# Autodesk Inventor assembly: DPLX_A005_Spark_Gap_Lab
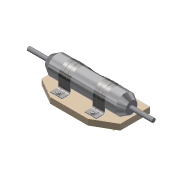
[picture p0: Inventor's stored thumbnail of the model, 180x180]
Saved by Autodesk Inventor 2018 (Build 220112000, 112)
## iProperties
Created: 2018-07-20
Part Number: DPLX_A005_Spark_Gap_Lab
Document SubType Name: Assembly
Designer: DPLXuser
Author: DPLXuser
## Documents named in this file (14)
- C:\Users\DPLXuser\Documents\GitHub\UMBC_DPLX_SPARK\SPARK CAD Files\DPLX_A005_Spark_Gap_Lab.iam
- C:\Users\DPLXuser\Documents\Michael Schwab\SPARK CAD Files\DPLX_P023 Spark Gap Shielding Bottom.ipt
- C:\Users\DPLXuser\Documents\Michael Schwab\SPARK CAD Files\DPLX_P022 Spark Gap Shielding Top.ipt
- C:\Users\DPLXuser\Documents\Michael Schwab\SPARK CAD Files\DPLX_P035 Spark Gap Shielding Middle.ipt
- C:\Users\DPLXuser\Documents\Michael Schwab\SPARK CAD Files\92010A787_PASSIVATED 18-8 SS PHILLIPS FLAT HEAD SCREW.ipt
- C:\Users\DPLXuser\Documents\Michael Schwab\SPARK CAD Files\92010A122_METRIC 18-8 SS FLAT HEAD PHIL MACHINE SCREW.ipt
- C:\Users\DPLXuser\Documents\Michael Schwab\SPARK CAD Files\9429T360_STEEL CLAMP.ipt
- C:\Users\DPLXuser\Documents\Michael Schwab\SPARK CAD Files\DPLX_P025_Quartz_Tube.ipt
- C:\Users\DPLXuser\Documents\Michael Schwab\SPARK CAD Files\DPLX_P007_Wire_Mesh_Sleeve_Spark_Gap.ipt
- C:\Users\DPLXuser\Documents\Michael Schwab\SPARK CAD Files\DPLX_P033_SG_Viton rubber Cover.ipt
- C:\Users\DPLXuser\Documents\Michael Schwab\SPARK CAD Files\DPLX_P015_Foil_Wrap_SG.ipt
- C:\Users\DPLXuser\Documents\Michael Schwab\SPARK CAD Files\DPLX_A001_revE_Electrode_assmMJS.iam
- C:\Users\DPLXuser\Documents\Michael Schwab\SPARK CAD Files\91828A211_TYPE 18-8 STAINLESS STEEL HEX NUT.ipt
- C:\Users\DPLXuser\Documents\Michael Schwab\SPARK CAD Files\DPLX_P010_Wire_Mesh_reducer_Spark_Gap.ipt
## Components (25 placed, 13 different names)
1. DPLX_P023 Spark Gap Shielding Bottom:1 — Mate:1, Mate:2
2. DPLX_P022 Spark Gap Shielding Top:1 — Mate:3, Mate:4, Mate:5, Mate:6, Insert:9, Insert:10, Insert:11, Insert:12
3. DPLX_P035 Spark Gap Shielding Middle:1 — Insert:1, Insert:2, Insert:3, Insert:4, Insert:5, Insert:6, Insert:7, Insert:8, Mate:1, Mate:2, Mate:3, Mate:4
4. 92010A787_PASSIVATED 18-8 SS PHILLIPS FLAT HEAD SCREW:1 — Insert:3
5. 92010A787_PASSIVATED 18-8 SS PHILLIPS FLAT HEAD SCREW:2 — Insert:4
6. 92010A787_PASSIVATED 18-8 SS PHILLIPS FLAT HEAD SCREW:3 — Insert:2
7. 92010A787_PASSIVATED 18-8 SS PHILLIPS FLAT HEAD SCREW:4 — Insert:1
8. 92010A122_METRIC 18-8 SS FLAT HEAD PHIL MACHINE SCREW:1 — Insert:6
9. 92010A122_METRIC 18-8 SS FLAT HEAD PHIL MACHINE SCREW:2 — Insert:8
10. 92010A122_METRIC 18-8 SS FLAT HEAD PHIL MACHINE SCREW:3 — Insert:5
11. 92010A122_METRIC 18-8 SS FLAT HEAD PHIL MACHINE SCREW:4 — Insert:7
12. 9429T360_STEEL CLAMP:1 — Mate:6, Insert:9, Insert:10, Insert:18, Insert:19, Insert:21
13. 9429T360_STEEL CLAMP:2 — Mate:5, Insert:11, Insert:12, Insert:20, Insert:22
14. DPLX_P025_Quartz_Tube:1 — Insert:13, Insert:16, Insert:17
15. DPLX_P007_Wire_Mesh_Sleeve_Spark_Gap:1 — Insert:15, Insert:18, Insert:23, Insert:24
16. DPLX_P033_SG_Viton rubber Cover:1 — Insert:13, Mate:7, Insert:14, Insert:15
17. DPLX_P015_Foil_Wrap_SG:1 — Mate:7, Insert:14
18. DPLX_A001_revE_Electrode_assmMJS:1 [sub-assembly] — Insert:16
19. DPLX_A001_revE_Electrode_assmMJS:2 [sub-assembly] — Insert:17
20. 91828A211_TYPE 18-8 STAINLESS STEEL HEX NUT:1 — Insert:22
21. 91828A211_TYPE 18-8 STAINLESS STEEL HEX NUT:2 — Insert:21
22. 91828A211_TYPE 18-8 STAINLESS STEEL HEX NUT:3 — Insert:20
23. 91828A211_TYPE 18-8 STAINLESS STEEL HEX NUT:4 — Insert:19
24. DPLX_P010_Wire_Mesh_reducer_Spark_Gap:1 — Insert:23
25. DPLX_P010_Wire_Mesh_reducer_Spark_Gap:2 — Insert:24
## Relationships (31: Insert 24, Mate 7)
- Insert:1: DPLX_P035 Spark Gap Shielding Middle:1 ↔ 92010A787_PASSIVATED 18-8 SS PHILLIPS FLAT HEAD SCREW:4
- Insert:2: DPLX_P035 Spark Gap Shielding Middle:1 ↔ 92010A787_PASSIVATED 18-8 SS PHILLIPS FLAT HEAD SCREW:3
- Insert:3: DPLX_P035 Spark Gap Shielding Middle:1 ↔ 92010A787_PASSIVATED 18-8 SS PHILLIPS FLAT HEAD SCREW:1
- Insert:4: DPLX_P035 Spark Gap Shielding Middle:1 ↔ 92010A787_PASSIVATED 18-8 SS PHILLIPS FLAT HEAD SCREW:2
- Insert:5: DPLX_P035 Spark Gap Shielding Middle:1 ↔ 92010A122_METRIC 18-8 SS FLAT HEAD PHIL MACHINE SCREW:3
- Insert:6: DPLX_P035 Spark Gap Shielding Middle:1 ↔ 92010A122_METRIC 18-8 SS FLAT HEAD PHIL MACHINE SCREW:1
- Insert:7: DPLX_P035 Spark Gap Shielding Middle:1 ↔ 92010A122_METRIC 18-8 SS FLAT HEAD PHIL MACHINE SCREW:4
- Insert:8: DPLX_P035 Spark Gap Shielding Middle:1 ↔ 92010A122_METRIC 18-8 SS FLAT HEAD PHIL MACHINE SCREW:2
- Mate:1: DPLX_P023 Spark Gap Shielding Bottom:1 ↔ DPLX_P035 Spark Gap Shielding Middle:1
- Mate:2: DPLX_P023 Spark Gap Shielding Bottom:1 ↔ DPLX_P035 Spark Gap Shielding Middle:1
- Mate:3: DPLX_P022 Spark Gap Shielding Top:1 ↔ DPLX_P035 Spark Gap Shielding Middle:1
- Mate:4: DPLX_P022 Spark Gap Shielding Top:1 ↔ DPLX_P035 Spark Gap Shielding Middle:1
- Mate:5: DPLX_P022 Spark Gap Shielding Top:1 ↔ 9429T360_STEEL CLAMP:2
- Mate:6: DPLX_P022 Spark Gap Shielding Top:1 ↔ 9429T360_STEEL CLAMP:1
- Insert:9: DPLX_P022 Spark Gap Shielding Top:1 ↔ 9429T360_STEEL CLAMP:1
- Insert:10: DPLX_P022 Spark Gap Shielding Top:1 ↔ 9429T360_STEEL CLAMP:1
- Insert:11: DPLX_P022 Spark Gap Shielding Top:1 ↔ 9429T360_STEEL CLAMP:2
- Insert:12: DPLX_P022 Spark Gap Shielding Top:1 ↔ 9429T360_STEEL CLAMP:2
- Insert:13: DPLX_P025_Quartz_Tube:1 ↔ DPLX_P033_SG_Viton rubber Cover:1
- Mate:7: DPLX_P033_SG_Viton rubber Cover:1 ↔ DPLX_P015_Foil_Wrap_SG:1
- Insert:14: DPLX_P033_SG_Viton rubber Cover:1 ↔ DPLX_P015_Foil_Wrap_SG:1
- Insert:15 (-5.08 mm): DPLX_P007_Wire_Mesh_Sleeve_Spark_Gap:1 ↔ DPLX_P033_SG_Viton rubber Cover:1
- Insert:16: DPLX_P025_Quartz_Tube:1 ↔ DPLX_A001_revE_Electrode_assmMJS:1
- Insert:17: DPLX_P025_Quartz_Tube:1 ↔ DPLX_A001_revE_Electrode_assmMJS:2
- Insert:18 (-17.78 mm): 9429T360_STEEL CLAMP:1 ↔ DPLX_P007_Wire_Mesh_Sleeve_Spark_Gap:1
- Insert:19: 9429T360_STEEL CLAMP:1 ↔ 91828A211_TYPE 18-8 STAINLESS STEEL HEX NUT:4
- Insert:20: 9429T360_STEEL CLAMP:2 ↔ 91828A211_TYPE 18-8 STAINLESS STEEL HEX NUT:3
- Insert:21: 9429T360_STEEL CLAMP:1 ↔ 91828A211_TYPE 18-8 STAINLESS STEEL HEX NUT:2
- Insert:22: 9429T360_STEEL CLAMP:2 ↔ 91828A211_TYPE 18-8 STAINLESS STEEL HEX NUT:1
- Insert:23: DPLX_P007_Wire_Mesh_Sleeve_Spark_Gap:1 ↔ DPLX_P010_Wire_Mesh_reducer_Spark_Gap:1
- Insert:24: DPLX_P007_Wire_Mesh_Sleeve_Spark_Gap:1 ↔ DPLX_P010_Wire_Mesh_reducer_Spark_Gap:2
